# Autodesk Inventor assembly: tarjeta
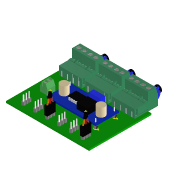
[picture p0: Inventor's stored thumbnail of the model, 180x180]
Saved by Autodesk Inventor 2022 (Build 260153000, 153)
## iProperties
Created: 2022-11-21
Part Number: tarjeta
Document SubType Name: Assembly
Designer: ferna
Author: ferna
## Documents named in this file (12)
- C:\Users\ferna\Documents\Bocas\Prototipo_09\Tarjeta Interrupciones\tarjeta.iam
- C:\Users\ferna\Documents\Bocas\Prototipo_09\Tarjeta Interrupciones\placa.ipt
- C:\Users\ferna\Downloads\shield_flautista (1)\1X03.ipt
- C:\Users\ferna\Downloads\shield_flautista (1)\1X01.ipt
- C:\Users\ferna\Downloads\shield_flautista (1)\TERMINAL-BLOCK-2-PIN-3.5MM-LONG-PAD.ipt
- C:\Users\ferna\Documents\Bocas\Prototipo_09\Tarjeta Interrupciones\dcdc.ipt
- C:\Users\ferna\Downloads\pluggable-terminal-connector-2-pin-1.snapshot.1\plugin_maleblock.ipt
- C:\Users\ferna\Downloads\pluggable-terminal-connector-2-pin-1.snapshot.1\Plugin_block.ipt
- C:\Users\ferna\Documents\Bocas\Prototipo_09\amci\conector_motores.ipt
- C:\Users\ferna\Downloads\pluggable-terminal-connector-2-pin-1.snapshot.1\Screw_Terminal.ipt
- C:\Users\ferna\Documents\Bocas\Prototipo_09\Tarjeta Interrupciones\tarjeta\AIP\Cable and Harness\tarjeta.Harness1.iam
- C:\Users\ferna\Documents\Bocas\Prototipo_09\arduino\concector_servos.ipt
## Components (43 placed, 11 different names)
1. placa:1 — Mate:1, Flush:1, Flush:2, Mate:2, Flush:3, Flush:4, Mate:4, Flush:7, Flush:8, Mate:6, Flush:11, Mate:9, Flush:16, Flush:17, Flush:18, Mate:10, Mate:49, Mate:50, Mate:51
2. TERMINAL-BLOCK-2-PIN-3.5MM-LONG-PAD:1 — Mate:4, Flush:7, Flush:8
3. dcdc:1 — Mate:3, Flush:5, Flush:6
4. plugin_maleblock:1 — Mate:5, Flush:9, Flush:10, Mate:6, Flush:16, Mate:12, Flush:27
5. plugin_maleblock:2 — Mate:5, Flush:9, Flush:10, Flush:11, Mate:44, Mate:45
6. plugin_maleblock:3 — Mate:11, Flush:26
7. plugin_maleblock:4 — Mate:9, Flush:17, Mate:12, Mate:42, Mate:43
8. plugin_maleblock:5 — Mate:10, Flush:25, Mate:41
9. plugin_maleblock:6 — Flush:18, Mate:11, Mate:40
10. Plugin_block:1 — Flush:19, Flush:20, Mate:13, Mate:14, Mate:15, Mate:20, Mate:21, Mate:40, Tangent:5
11. conector_motores:1 — Mate:46, Tangent:1, Tangent:2
12. Plugin_block:2 — Flush:19, Flush:20, Mate:13, Mate:16, Mate:17, Mate:18, Mate:19, Flush:25, Mate:41, Mate:48, Tangent:4
13. Screw_Terminal:1 — Mate:14, Mate:21
14. Screw_Terminal:2 — Mate:15, Mate:20
15. Screw_Terminal:3 — Mate:16, Mate:19
16. Screw_Terminal:4 — Mate:17, Mate:18
17. Plugin_block:3 — Mate:44, Mate:45, Tangent:2
18. Plugin_block:4 — Flush:27, Mate:46, Tangent:1
19. Screw_Terminal:5
20. Screw_Terminal:6
21. Screw_Terminal:7
22. Screw_Terminal:8
23. Plugin_block:5 — Mate:42, Tangent:6
24. Plugin_block:6 — Flush:26, Mate:43, Mate:47, Tangent:3
25. Screw_Terminal:9
26. Screw_Terminal:10
27. Screw_Terminal:11
28. Screw_Terminal:12
29. conector_motores:2 — Mate:48, Tangent:4, Tangent:5
30. conector_motores:3 — Mate:47, Tangent:3, Tangent:6
31. Harness1 [sub-assembly]
32. concector_servos:1 — Mate:53, Flush:30, Flush:31
33. concector_servos:2 — Flush:28, Mate:52, Flush:29
34. 1X03:1 — Mate:1, Flush:1, Flush:2, Flush:28, Mate:52, Flush:29
35. 1X03:2
36. 1X03:3
37. 1X03:4 — Mate:53, Flush:30, Flush:31
38. 1X03:5
39. 1X03:6
40. 1X01:1 — Mate:2, Flush:3, Flush:4, Mate:3
41. 1X01:2
42. 1X01:3 — Flush:5
43. 1X01:4 — Flush:6
## Component patterns: (6 elements, first: 1X03:1), (4 elements, first: 1X01:1)
## Relationships (90: Mate 53, Flush 31, Tangent 6)
- Mate:1: placa:1 ↔ 1X03:1
- Flush:1 (3.75 mm): placa:1 ↔ 1X03:1
- Flush:2 (-9.47 mm): placa:1 ↔ 1X03:1
- Mate:2: placa:1 ↔ 1X01:1
- Flush:3 (12 mm): placa:1 ↔ 1X01:1
- Flush:4 (17.8 mm): placa:1 ↔ 1X01:1
- Mate:3 (1 mm): dcdc:1 ↔ 1X01:1
- Flush:5 (-0.74 mm): dcdc:1 ↔ 1X01:3
- Flush:6 (-0.74 mm): dcdc:1 ↔ 1X01:4
- Mate:4: placa:1 ↔ TERMINAL-BLOCK-2-PIN-3.5MM-LONG-PAD:1
- Flush:7 (22.85 mm): placa:1 ↔ TERMINAL-BLOCK-2-PIN-3.5MM-LONG-PAD:1
- Flush:8 (-7.7 mm): placa:1 ↔ TERMINAL-BLOCK-2-PIN-3.5MM-LONG-PAD:1
- Mate:5: plugin_maleblock:1 ↔ plugin_maleblock:2
- Flush:9: plugin_maleblock:1 ↔ plugin_maleblock:2
- Flush:10: plugin_maleblock:1 ↔ plugin_maleblock:2
- Mate:6: placa:1 ↔ plugin_maleblock:1
- Flush:11 (3.6 mm): placa:1 ↔ plugin_maleblock:2
- [Mate]: plugin_maleblock:3 ↔ plugin_maleblock:4
- [Flush]: plugin_maleblock:3 ↔ plugin_maleblock:4
- [Flush]: plugin_maleblock:3 ↔ plugin_maleblock:4
- [Mate]: plugin_maleblock:5 ↔ plugin_maleblock:6
- [Flush]: plugin_maleblock:5 ↔ plugin_maleblock:6
- [Flush]: plugin_maleblock:5 ↔ plugin_maleblock:6
- Mate:9: placa:1 ↔ plugin_maleblock:4
- Flush:16: placa:1 ↔ plugin_maleblock:1
- Flush:17: placa:1 ↔ plugin_maleblock:4
- Flush:18: placa:1 ↔ plugin_maleblock:6
- Mate:10: placa:1 ↔ plugin_maleblock:5
- Mate:11 (3 mm): plugin_maleblock:3 ↔ plugin_maleblock:6
- Mate:12 (3 mm): plugin_maleblock:1 ↔ plugin_maleblock:4
- Flush:19: Plugin_block:1 ↔ Plugin_block:2
- Flush:20: Plugin_block:1 ↔ Plugin_block:2
- Mate:13: Plugin_block:1 ↔ Plugin_block:2
- Mate:14: Plugin_block:1 ↔ Screw_Terminal:1
- Mate:15: Plugin_block:1 ↔ Screw_Terminal:2
- Mate:16: Plugin_block:2 ↔ Screw_Terminal:3
- Mate:17: Plugin_block:2 ↔ Screw_Terminal:4
- Mate:18: Plugin_block:2 ↔ Screw_Terminal:4
- Mate:19: Plugin_block:2 ↔ Screw_Terminal:3
- Mate:20: Plugin_block:1 ↔ Screw_Terminal:2
- Mate:21: Plugin_block:1 ↔ Screw_Terminal:1
- [Flush]: Plugin_block:3 ↔ Plugin_block:4
- [Flush]: Plugin_block:3 ↔ Plugin_block:4
- [Mate]: Plugin_block:3 ↔ Plugin_block:4
- [Mate]: Plugin_block:3 ↔ Screw_Terminal:5
- [Mate]: Plugin_block:3 ↔ Screw_Terminal:6
- [Mate]: Plugin_block:4 ↔ Screw_Terminal:7
- [Mate]: Plugin_block:4 ↔ Screw_Terminal:8
- [Mate]: Plugin_block:4 ↔ Screw_Terminal:8
- [Mate]: Plugin_block:4 ↔ Screw_Terminal:7
- [Mate]: Plugin_block:3 ↔ Screw_Terminal:6
- [Mate]: Plugin_block:3 ↔ Screw_Terminal:5
- [Flush]: Plugin_block:5 ↔ Plugin_block:6
- [Flush]: Plugin_block:5 ↔ Plugin_block:6
- [Mate]: Plugin_block:5 ↔ Plugin_block:6
- [Mate]: Plugin_block:5 ↔ Screw_Terminal:9
- [Mate]: Plugin_block:5 ↔ Screw_Terminal:10
- [Mate]: Plugin_block:6 ↔ Screw_Terminal:11
- [Mate]: Plugin_block:6 ↔ Screw_Terminal:12
- [Mate]: Plugin_block:6 ↔ Screw_Terminal:12
- [Mate]: Plugin_block:6 ↔ Screw_Terminal:11
- [Mate]: Plugin_block:5 ↔ Screw_Terminal:10
- [Mate]: Plugin_block:5 ↔ Screw_Terminal:9
- Mate:40: plugin_maleblock:6 ↔ Plugin_block:1
- Flush:25: plugin_maleblock:5 ↔ Plugin_block:2
- Mate:41: plugin_maleblock:5 ↔ Plugin_block:2
- Mate:42: plugin_maleblock:4 ↔ Plugin_block:5
- Flush:26: plugin_maleblock:3 ↔ Plugin_block:6
- Mate:43: plugin_maleblock:4 ↔ Plugin_block:6
- Flush:27: plugin_maleblock:1 ↔ Plugin_block:4
- Mate:44: plugin_maleblock:2 ↔ Plugin_block:3
- Mate:45: plugin_maleblock:2 ↔ Plugin_block:3
- Mate:46 (10 mm): conector_motores:1 ↔ Plugin_block:4
- Tangent:1: conector_motores:1 ↔ Plugin_block:4
- Tangent:2 (-2 mm): conector_motores:1 ↔ Plugin_block:3
- Mate:47 (10 mm): Plugin_block:6 ↔ conector_motores:3
- Mate:48 (10 mm): Plugin_block:2 ↔ conector_motores:2
- Tangent:3: Plugin_block:6 ↔ conector_motores:3
- Tangent:4: Plugin_block:2 ↔ conector_motores:2
- Tangent:5 (-2 mm): Plugin_block:1 ↔ conector_motores:2
- Tangent:6 (-2 mm): Plugin_block:5 ↔ conector_motores:3
- Mate:49: placa:1
- Mate:50: placa:1
- Mate:51: placa:1
- Flush:28: concector_servos:2 ↔ 1X03:1
- Mate:52: concector_servos:2 ↔ 1X03:1
- Flush:29: concector_servos:2 ↔ 1X03:1
- Mate:53: concector_servos:1 ↔ 1X03:4
- Flush:30: concector_servos:1 ↔ 1X03:4
- Flush:31: concector_servos:1 ↔ 1X03:4
## Named parameters: d25_d20 = 0 mm, d26_d21 = 0 mm, d27_d22 = 0 mm, d28_d20 = 0 mm, d29_d21 = 0 mm, d30_d22 = 0 mm, d55_d47 = 0 mm, d56_d48 = 0 mm, d57_d49 = 0 mm, d58_d50 = 0 mm, d59_d51 = 0 mm, d60_d52 = 0 mm, d61_d53 = 0 mm, d62_d54 = 0 mm, d63_d38 = 0 mm, d64_d39 = 0 mm, d65_d40 = 0 mm, d66_d47 = 0 mm, d67_d48 = 0 mm, d68_d49 = 0 mm, d69_d50 = 0 mm, d70_d51 = 0 mm, d71_d52 = 0 mm, d72_d53 = 0 mm, d73_d54 = 0 mm, d74_d38 = 0 mm, d75_d39 = 0 mm, d76_d40 = 0 mm
